# Autodesk Inventor assembly: Ensamblaje3
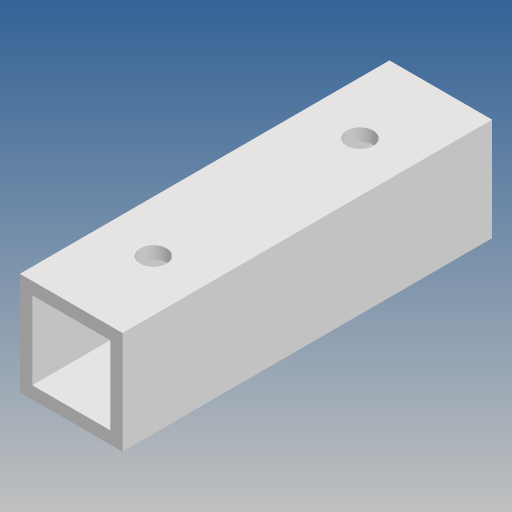
[picture p0: Inventor's stored thumbnail of the model, 512x512]
Saved by Autodesk Inventor 2024 (Build 280153000, 153)
## iProperties
Created: 2024-05-31
Part Number: Ensamblaje3
Document SubType Name: Assembly
Designer: Pablo
Author: Pablo
## Documents named in this file (3)
- D:\Users\Pablo\Desktop\UVG\otros\TesisM\Ensamblaje3.iam
- D:\Users\Pablo\Desktop\UVG\otros\TesisM\Pieza8.ipt
- D:\Users\Pablo\Desktop\UVG\otros\TesisM\Pieza9.ipt
## Components (4 placed, 2 different names)
1. Pieza8:1 — Nivelación:2, Nivelación:3, Nivelación:4, Nivelación:9, Nivelación:11, Nivelación:12
2. Pieza8:2 — Nivelación:6, Nivelación:7, Nivelación:8, Nivelación:10
3. Pieza9:1 — Nivelación:4, Nivelación:11, Nivelación:12
4. Pieza9:2 — Nivelación:2, Nivelación:3, Nivelación:6, Nivelación:7, Nivelación:8, Nivelación:9, Nivelación:10
## Relationships (10: Flush 10)
- Nivelación:2 [Flush]: Pieza8:1 ↔ Pieza9:2
- Nivelación:3 [Flush]: Pieza8:1 ↔ Pieza9:2
- Nivelación:4 [Flush]: Pieza8:1 ↔ Pieza9:1
- Nivelación:6 [Flush]: Pieza8:2 ↔ Pieza9:2
- Nivelación:7 [Flush]: Pieza8:2 ↔ Pieza9:2
- Nivelación:8 [Flush]: Pieza8:2 ↔ Pieza9:2
- Nivelación:9 [Flush]: Pieza8:1 ↔ Pieza9:2
- Nivelación:10 [Flush]: Pieza8:2 ↔ Pieza9:2
- Nivelación:11 [Flush]: Pieza8:1 ↔ Pieza9:1
- Nivelación:12 [Flush]: Pieza8:1 ↔ Pieza9:1
